# Autodesk Inventor assembly: WallBody
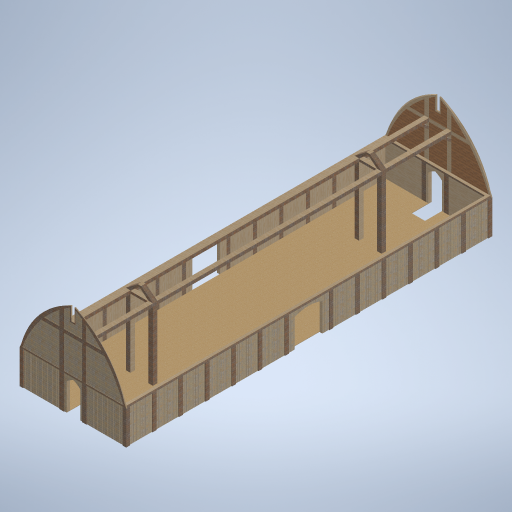
[picture p0: Inventor's stored thumbnail of the model, 512x512]
Saved by Autodesk Inventor 2024.2 (Build 282272000, 272)
## iProperties
Created: 2024-05-21
Part Number: WallBody
Document SubType Name: Assembly
Designer: LOSTER_1
Author: LOSTER_1
## Documents named in this file (62)
- C:\Users\LOSTER_1\OneDrive\桌面\school\senior\Inventor_Project\WALL\WallBody.iam
- C:\Users\LOSTER_1\OneDrive\桌面\school\senior\Inventor_Project\WALL\curve_front_wall_frame.ipt
- C:\Users\LOSTER_1\OneDrive\桌面\school\senior\Inventor_Project\WALL\top_wall_frame.ipt
- C:\Users\LOSTER_1\OneDrive\桌面\school\senior\Inventor_Project\WALL\front_wall_block01.ipt
- C:\Users\LOSTER_1\OneDrive\桌面\school\senior\Inventor_Project\WALL\front_wall_block02.ipt
- C:\Users\LOSTER_1\OneDrive\桌面\school\senior\Inventor_Project\WALL\front_wall_block03.ipt
- C:\Users\LOSTER_1\OneDrive\桌面\school\senior\Inventor_Project\WALL\front_wall_block04.ipt
- C:\Users\LOSTER_1\OneDrive\桌面\school\senior\Inventor_Project\WALL\front_wall_block01_MIR.ipt
- C:\Users\LOSTER_1\OneDrive\桌面\school\senior\Inventor_Project\WALL\front_wall_block02_MIR.ipt
- C:\Users\LOSTER_1\OneDrive\桌面\school\senior\Inventor_Project\WALL\front_wall_block03_MIR.ipt
- C:\Users\LOSTER_1\OneDrive\桌面\school\senior\Inventor_Project\WALL\front_wall_block04_MIR.ipt
- C:\Users\LOSTER_1\OneDrive\桌面\school\senior\Inventor_Project\WALL\curve_front_wall_frame_MIR.ipt
- C:\Users\LOSTER_1\OneDrive\桌面\school\senior\Inventor_Project\WALL\front_wall_block01_MIR1.ipt
- C:\Users\LOSTER_1\OneDrive\桌面\school\senior\Inventor_Project\WALL\front_wall_block02_MIR1.ipt
- C:\Users\LOSTER_1\OneDrive\桌面\school\senior\Inventor_Project\WALL\front_wall_block03_MIR1.ipt
- C:\Users\LOSTER_1\OneDrive\桌面\school\senior\Inventor_Project\WALL\front_wall_block04_MIR1.ipt
- C:\Users\LOSTER_1\OneDrive\桌面\school\senior\Inventor_Project\WALL\front_wall_block01_MIR_MIR.ipt
- C:\Users\LOSTER_1\OneDrive\桌面\school\senior\Inventor_Project\WALL\front_wall_block02_MIR_MIR.ipt
- C:\Users\LOSTER_1\OneDrive\桌面\school\senior\Inventor_Project\WALL\front_wall_block03_MIR_MIR.ipt
- C:\Users\LOSTER_1\OneDrive\桌面\school\senior\Inventor_Project\WALL\front_wall_block04_MIR_MIR.ipt
- C:\Users\LOSTER_1\OneDrive\桌面\school\senior\Inventor_Project\WALL\support_frame_01.ipt
- C:\Users\LOSTER_1\OneDrive\桌面\school\senior\Inventor_Project\WALL\support_frame_02.ipt
- C:\Users\LOSTER_1\OneDrive\桌面\school\senior\Inventor_Project\WALL\support_frame_02_MIR.ipt
- C:\Users\LOSTER_1\OneDrive\桌面\school\senior\Inventor_Project\WALL\support_frame_01_MIR.ipt
- C:\Users\LOSTER_1\OneDrive\桌面\school\senior\Inventor_Project\WALL\support_column_01.ipt
- C:\Users\LOSTER_1\OneDrive\桌面\school\senior\Inventor_Project\WALL\support_column_01_MIR.ipt
- C:\Users\LOSTER_1\OneDrive\桌面\school\senior\Inventor_Project\WALL\support_column_01_MIR1.ipt
- C:\Users\LOSTER_1\OneDrive\桌面\school\senior\Inventor_Project\WALL\support_column_01_MIR_MIR.ipt
- C:\Users\LOSTER_1\OneDrive\桌面\school\senior\Inventor_Project\WALL\support_column_02.ipt
- C:\Users\LOSTER_1\OneDrive\桌面\school\senior\Inventor_Project\WALL\support_column_02_MIR.ipt
- C:\Users\LOSTER_1\OneDrive\桌面\school\senior\Inventor_Project\WALL\support_column_02_MIR1.ipt
- C:\Users\LOSTER_1\OneDrive\桌面\school\senior\Inventor_Project\WALL\support_column_02_MIR_MIR.ipt
- C:\Users\LOSTER_1\OneDrive\桌面\school\senior\Inventor_Project\WALL\ribs\frame_rib_01.ipt
- C:\Users\LOSTER_1\OneDrive\桌面\school\senior\Inventor_Project\WALL\ribs\frame_rib_01_MIR.ipt
- C:\Users\LOSTER_1\OneDrive\桌面\school\senior\Inventor_Project\WALL\ribs\frame_rib_01_MIR1.ipt
- C:\Users\LOSTER_1\OneDrive\桌面\school\senior\Inventor_Project\WALL\ribs\frame_rib_01_MIR_MIR.ipt
- C:\Users\LOSTER_1\OneDrive\桌面\school\senior\Inventor_Project\WALL\ribs\frame_rib_02.ipt
- C:\Users\LOSTER_1\OneDrive\桌面\school\senior\Inventor_Project\WALL\ribs\frame_rib_02_MIR.ipt
- C:\Users\LOSTER_1\OneDrive\桌面\school\senior\Inventor_Project\WALL\ribs\frame_rib_02_MIR1.ipt
- C:\Users\LOSTER_1\OneDrive\桌面\school\senior\Inventor_Project\WALL\ribs\frame_rib_02_MIR_MIR.ipt
- C:\Users\LOSTER_1\OneDrive\桌面\school\senior\Inventor_Project\WALL\support_frame_03.ipt
- C:\Users\LOSTER_1\OneDrive\桌面\school\senior\Inventor_Project\WALL\support_frame_03_MIR.ipt
- C:\Users\LOSTER_1\OneDrive\桌面\school\senior\Inventor_Project\WALL\support_frame_03_MIR1.ipt
- C:\Users\LOSTER_1\OneDrive\桌面\school\senior\Inventor_Project\WALL\support_frame_03_MIR_MIR.ipt
- C:\Users\LOSTER_1\OneDrive\桌面\school\senior\Inventor_Project\WALL\normalized_wall_block\side_wall_block_01.ipt
- C:\Users\LOSTER_1\OneDrive\桌面\school\senior\Inventor_Project\WALL\normalized_wall_block\side_wall_block_02.ipt
- C:\Users\LOSTER_1\OneDrive\桌面\school\senior\Inventor_Project\WALL\normalized_wall_block\side_wall_block_01_MIR.ipt
- C:\Users\LOSTER_1\OneDrive\桌面\school\senior\Inventor_Project\WALL\support_column_01_MIR2.ipt
- C:\Users\LOSTER_1\OneDrive\桌面\school\senior\Inventor_Project\WALL\normalized_wall_block\side_wall_block_02_MIR.ipt
- C:\Users\LOSTER_1\OneDrive\桌面\school\senior\Inventor_Project\WALL\normalized_wall_block\side_wall_block_01_MIR1.ipt
- C:\Users\LOSTER_1\OneDrive\桌面\school\senior\Inventor_Project\WALL\support_column_01_MIR3.ipt
- C:\Users\LOSTER_1\OneDrive\桌面\school\senior\Inventor_Project\WALL\normalized_wall_block\side_wall_block_02_MIR1.ipt
- C:\Users\LOSTER_1\OneDrive\桌面\school\senior\Inventor_Project\WALL\normalized_wall_block\side_wall_block_01_MIR_MIR.ipt
- C:\Users\LOSTER_1\OneDrive\桌面\school\senior\Inventor_Project\WALL\support_column_01_MIR2_MIR.ipt
- C:\Users\LOSTER_1\OneDrive\桌面\school\senior\Inventor_Project\WALL\normalized_wall_block\side_wall_block_02_MIR_MIR.ipt
- C:\Users\LOSTER_1\OneDrive\桌面\school\senior\Inventor_Project\WALL\front_wall_block05.ipt
- C:\Users\LOSTER_1\OneDrive\桌面\school\senior\Inventor_Project\WALL\front_wall_block05_MIR.ipt
- C:\Users\LOSTER_1\OneDrive\桌面\school\senior\Inventor_Project\WALL\front_wall_block05_MIR1.ipt
- C:\Users\LOSTER_1\OneDrive\桌面\school\senior\Inventor_Project\WALL\front_wall_block05_MIR_MIR.ipt
- C:\Users\LOSTER_1\OneDrive\桌面\school\senior\Inventor_Project\WALL\front_wall_block06.ipt
- C:\Users\LOSTER_1\OneDrive\桌面\school\senior\Inventor_Project\FLOOR\inside_floor.ipt
- C:\Users\LOSTER_1\OneDrive\桌面\school\senior\Inventor_Project\WALL\front_wall_block06_MIR1.ipt
## Components (102 placed, 61 different names)
1. curve_front_wall_frame:1 — Flush:1, Mate:1, Mate:2, Flush:2, Mate:3, Mate:4, Mate:5, Mate:7, Mate:8, Mate:9, Mate:18
2. top_wall_frame:1 — Mate:1, Mate:2, Mate:6, Mate:10, Mate:24, Mate:35, Mate:36, Mate:37, Mate:39, Mate:41, Mate:43, Mate:45, Mate:47, Mate:49, Mate:51, Mate:53, Mate:55, Mate:57, Mate:59, Mate:97, Mate:99
3. front_wall_block01:1 — Mate:3, Mate:4
4. front_wall_block02:1 — Mate:5, Mate:6
5. front_wall_block03:1 — Mate:7, Mate:8
6. front_wall_block04:1 — Mate:9, Mate:10
7. front_wall_block01_MIR:1
8. front_wall_block02_MIR:1 — Mate:19, Mate:20
9. front_wall_block03_MIR:1
10. front_wall_block04_MIR:1
11. curve_front_wall_frame_MIR:1 — Mate:11, Mate:12, Mate:13, Mate:14, Mate:15, Mate:16, Mate:17, Mate:25, Mate:26, Mate:27, Mate:28
12. front_wall_block01_MIR1:1 — Mate:12, Mate:13
13. front_wall_block02_MIR1:1 — Mate:14
14. front_wall_block03_MIR1:1 — Mate:15, Mate:16
15. front_wall_block04_MIR1:1 — Mate:17
16. front_wall_block01_MIR_MIR:1
17. front_wall_block02_MIR_MIR:1
18. front_wall_block03_MIR_MIR:1
19. front_wall_block04_MIR_MIR:1
20. support_frame_01:1 — Mate:18, Mate:19, Mate:20, Mate:21, Mate:22, Mate:23
21. support_frame_02:1 — Mate:21, Mate:22, Mate:23
22. support_frame_02_MIR:1
23. support_frame_01_MIR:1 — Mate:29, Mate:30, Mate:31, Mate:32, Mate:33, Mate:34
24. support_column_01:1 — Mate:24, Mate:25, Mate:26
25. support_column_01_MIR:1
26. support_column_01_MIR1:1
27. support_column_01_MIR_MIR:1
28. support_column_02:1 — Mate:27, Mate:28, Mate:100
29. support_column_02_MIR:1
30. support_column_02_MIR1:1
31. support_column_02_MIR_MIR:1
32. frame_rib_01:1 — Mate:29, Mate:30
33. frame_rib_01_MIR:1
34. frame_rib_01_MIR1:1
35. frame_rib_01_MIR_MIR:1
36. frame_rib_02:1 — Mate:31, Mate:32
37. frame_rib_02_MIR:1
38. frame_rib_02_MIR1:1
39. frame_rib_02_MIR_MIR:1
40. support_frame_03:1 — Mate:33, Mate:34
41. support_frame_03_MIR:1
42. support_frame_03_MIR1:1
43. support_frame_03_MIR_MIR:1
44. side_wall_block_01:1 — Mate:35, Mate:36, Mate:38, Mate:98
45. support_column_01:2 — Mate:37, Mate:38, Mate:40
46. side_wall_block_01:2 — Mate:39, Mate:40, Mate:42
47. support_column_01:3 — Mate:41, Mate:42, Mate:44
48. side_wall_block_01:3 — Mate:43, Mate:44, Mate:46
49. support_column_01:4 — Mate:45, Mate:46, Mate:48
50. side_wall_block_01:4 — Mate:47, Mate:48, Mate:50
51. support_column_01:5 — Mate:49, Mate:50, Mate:52
52. side_wall_block_01:5 — Mate:51, Mate:52, Mate:54
53. support_column_01:6 — Mate:53, Mate:54, Mate:56
54. side_wall_block_01:6 — Mate:55, Mate:56, Mate:58
55. support_column_01:7 — Mate:57, Mate:58, Mate:60
56. side_wall_block_02:1 — Mate:59, Mate:60
57. side_wall_block_01_MIR:1 — Mate:61
58. support_column_01_MIR2:1 — Mate:61, Mate:62
59. side_wall_block_01_MIR:2 — Mate:62, Mate:63
60. support_column_01_MIR2:2 — Mate:63, Mate:64
61. side_wall_block_01_MIR:3 — Mate:64, Mate:65
62. support_column_01_MIR2:3 — Mate:65, Mate:66
63. side_wall_block_01_MIR:4 — Mate:66, Mate:67
64. support_column_01_MIR2:4 — Mate:67, Mate:68
65. side_wall_block_01_MIR:5 — Mate:68, Mate:69
66. support_column_01_MIR2:5 — Mate:69, Mate:70
67. side_wall_block_01_MIR:6 — Mate:70, Mate:71
68. support_column_01_MIR2:6 — Mate:71, Mate:72
69. side_wall_block_02_MIR:1 — Mate:72
70. side_wall_block_01_MIR1:1 — Mate:73
71. support_column_01_MIR3:1 — Mate:73, Mate:74
72. side_wall_block_01_MIR1:2 — Mate:74, Mate:75
73. support_column_01_MIR3:2 — Mate:75, Mate:76
74. side_wall_block_01_MIR1:3 — Mate:76, Mate:77
75. support_column_01_MIR3:3 — Mate:77, Mate:78
76. side_wall_block_01_MIR1:4 — Mate:78, Mate:79
77. support_column_01_MIR3:4 — Mate:79, Mate:80
78. side_wall_block_01_MIR1:5 — Mate:80, Mate:81
79. support_column_01_MIR3:5 — Mate:81, Mate:82
80. side_wall_block_01_MIR1:6 — Mate:82, Mate:83
81. support_column_01_MIR3:6 — Mate:83, Mate:84
82. side_wall_block_02_MIR1:1 — Mate:84
83. side_wall_block_01_MIR_MIR:1 — Mate:85
84. support_column_01_MIR2_MIR:1 — Mate:85, Mate:86
85. side_wall_block_01_MIR_MIR:2 — Mate:86, Mate:87
86. support_column_01_MIR2_MIR:2 — Mate:87, Mate:88
87. side_wall_block_01_MIR_MIR:3 — Mate:88, Mate:89
88. support_column_01_MIR2_MIR:3 — Mate:89, Mate:90
89. side_wall_block_01_MIR_MIR:4 — Mate:90, Mate:91
90. support_column_01_MIR2_MIR:4 — Mate:91, Mate:92
91. side_wall_block_01_MIR_MIR:5 — Mate:92, Mate:93
92. support_column_01_MIR2_MIR:5 — Mate:93, Mate:94
93. side_wall_block_01_MIR_MIR:6 — Mate:94, Mate:95
94. support_column_01_MIR2_MIR:6 — Mate:95, Mate:96
95. side_wall_block_02_MIR_MIR:1 — Mate:96
96. front_wall_block05:1 — Mate:97, Mate:98
97. front_wall_block05_MIR:1 — Mate:101
98. front_wall_block05_MIR1:1
99. front_wall_block05_MIR_MIR:1
100. front_wall_block06:1 — Mate:99, Mate:100
101. inside_floor:1 — Mate:101
102. front_wall_block06_MIR1:1
## Relationships (103: Mate 101, Flush 2)
- Flush:1 (16151 mm): curve_front_wall_frame:1
- Mate:1: curve_front_wall_frame:1 ↔ top_wall_frame:1
- Mate:2: curve_front_wall_frame:1 ↔ top_wall_frame:1
- Flush:2 (150 mm): curve_front_wall_frame:1
- Mate:3: curve_front_wall_frame:1 ↔ front_wall_block01:1
- Mate:4: curve_front_wall_frame:1 ↔ front_wall_block01:1
- Mate:5: curve_front_wall_frame:1 ↔ front_wall_block02:1
- Mate:6: top_wall_frame:1 ↔ front_wall_block02:1
- Mate:7: curve_front_wall_frame:1 ↔ front_wall_block03:1
- Mate:8: curve_front_wall_frame:1 ↔ front_wall_block03:1
- Mate:9: curve_front_wall_frame:1 ↔ front_wall_block04:1
- Mate:10: top_wall_frame:1 ↔ front_wall_block04:1
- Mate:11 (16151 mm): curve_front_wall_frame_MIR:1
- Mate:12: curve_front_wall_frame_MIR:1 ↔ front_wall_block01_MIR1:1
- Mate:13: curve_front_wall_frame_MIR:1 ↔ front_wall_block01_MIR1:1
- Mate:14: curve_front_wall_frame_MIR:1 ↔ front_wall_block02_MIR1:1
- Mate:15: curve_front_wall_frame_MIR:1 ↔ front_wall_block03_MIR1:1
- Mate:16: curve_front_wall_frame_MIR:1 ↔ front_wall_block03_MIR1:1
- Mate:17: curve_front_wall_frame_MIR:1 ↔ front_wall_block04_MIR1:1
- Mate:18: curve_front_wall_frame:1 ↔ support_frame_01:1
- Mate:19: front_wall_block02_MIR:1 ↔ support_frame_01:1
- Mate:20: front_wall_block02_MIR:1 ↔ support_frame_01:1
- Mate:21: support_frame_01:1 ↔ support_frame_02:1
- Mate:22: support_frame_01:1 ↔ support_frame_02:1
- Mate:23: support_frame_01:1 ↔ support_frame_02:1
- Mate:24: top_wall_frame:1 ↔ support_column_01:1
- Mate:25: curve_front_wall_frame_MIR:1 ↔ support_column_01:1
- Mate:26: curve_front_wall_frame_MIR:1 ↔ support_column_01:1
- Mate:27: curve_front_wall_frame_MIR:1 ↔ support_column_02:1
- Mate:28: curve_front_wall_frame_MIR:1 ↔ support_column_02:1
- Mate:29: support_frame_01_MIR:1 ↔ frame_rib_01:1
- Mate:30: support_frame_01_MIR:1 ↔ frame_rib_01:1
- Mate:31: support_frame_01_MIR:1 ↔ frame_rib_02:1
- Mate:32: support_frame_01_MIR:1 ↔ frame_rib_02:1
- Mate:33: support_frame_01_MIR:1 ↔ support_frame_03:1
- Mate:34: support_frame_01_MIR:1 ↔ support_frame_03:1
- Mate:35: top_wall_frame:1 ↔ side_wall_block_01:1
- Mate:36: top_wall_frame:1 ↔ side_wall_block_01:1
- Mate:37: top_wall_frame:1 ↔ support_column_01:2
- Mate:38: side_wall_block_01:1 ↔ support_column_01:2
- Mate:39: top_wall_frame:1 ↔ side_wall_block_01:2
- Mate:40: support_column_01:2 ↔ side_wall_block_01:2
- Mate:41: top_wall_frame:1 ↔ support_column_01:3
- Mate:42: side_wall_block_01:2 ↔ support_column_01:3
- Mate:43: top_wall_frame:1 ↔ side_wall_block_01:3
- Mate:44: support_column_01:3 ↔ side_wall_block_01:3
- Mate:45: top_wall_frame:1 ↔ support_column_01:4
- Mate:46: side_wall_block_01:3 ↔ support_column_01:4
- Mate:47: top_wall_frame:1 ↔ side_wall_block_01:4
- Mate:48: support_column_01:4 ↔ side_wall_block_01:4
- Mate:49: top_wall_frame:1 ↔ support_column_01:5
- Mate:50: side_wall_block_01:4 ↔ support_column_01:5
- Mate:51: top_wall_frame:1 ↔ side_wall_block_01:5
- Mate:52: support_column_01:5 ↔ side_wall_block_01:5
- Mate:53: top_wall_frame:1 ↔ support_column_01:6
- Mate:54: side_wall_block_01:5 ↔ support_column_01:6
- Mate:55: top_wall_frame:1 ↔ side_wall_block_01:6
- Mate:56: support_column_01:6 ↔ side_wall_block_01:6
- Mate:57: top_wall_frame:1 ↔ support_column_01:7
- Mate:58: side_wall_block_01:6 ↔ support_column_01:7
- Mate:59: top_wall_frame:1 ↔ side_wall_block_02:1
- Mate:60: support_column_01:7 ↔ side_wall_block_02:1
- Mate:61: side_wall_block_01_MIR:1 ↔ support_column_01_MIR2:1
- Mate:62: support_column_01_MIR2:1 ↔ side_wall_block_01_MIR:2
- Mate:63: side_wall_block_01_MIR:2 ↔ support_column_01_MIR2:2
- Mate:64: support_column_01_MIR2:2 ↔ side_wall_block_01_MIR:3
- Mate:65: side_wall_block_01_MIR:3 ↔ support_column_01_MIR2:3
- Mate:66: support_column_01_MIR2:3 ↔ side_wall_block_01_MIR:4
- Mate:67: side_wall_block_01_MIR:4 ↔ support_column_01_MIR2:4
- Mate:68: support_column_01_MIR2:4 ↔ side_wall_block_01_MIR:5
- Mate:69: side_wall_block_01_MIR:5 ↔ support_column_01_MIR2:5
- Mate:70: support_column_01_MIR2:5 ↔ side_wall_block_01_MIR:6
- Mate:71: side_wall_block_01_MIR:6 ↔ support_column_01_MIR2:6
- Mate:72: support_column_01_MIR2:6 ↔ side_wall_block_02_MIR:1
- Mate:73: side_wall_block_01_MIR1:1 ↔ support_column_01_MIR3:1
- Mate:74: support_column_01_MIR3:1 ↔ side_wall_block_01_MIR1:2
- Mate:75: side_wall_block_01_MIR1:2 ↔ support_column_01_MIR3:2
- Mate:76: support_column_01_MIR3:2 ↔ side_wall_block_01_MIR1:3
- Mate:77: side_wall_block_01_MIR1:3 ↔ support_column_01_MIR3:3
- Mate:78: support_column_01_MIR3:3 ↔ side_wall_block_01_MIR1:4
- Mate:79: side_wall_block_01_MIR1:4 ↔ support_column_01_MIR3:4
- Mate:80: support_column_01_MIR3:4 ↔ side_wall_block_01_MIR1:5
- Mate:81: side_wall_block_01_MIR1:5 ↔ support_column_01_MIR3:5
- Mate:82: support_column_01_MIR3:5 ↔ side_wall_block_01_MIR1:6
- Mate:83: side_wall_block_01_MIR1:6 ↔ support_column_01_MIR3:6
- Mate:84: support_column_01_MIR3:6 ↔ side_wall_block_02_MIR1:1
- Mate:85: side_wall_block_01_MIR_MIR:1 ↔ support_column_01_MIR2_MIR:1
- Mate:86: support_column_01_MIR2_MIR:1 ↔ side_wall_block_01_MIR_MIR:2
- Mate:87: side_wall_block_01_MIR_MIR:2 ↔ support_column_01_MIR2_MIR:2
- Mate:88: support_column_01_MIR2_MIR:2 ↔ side_wall_block_01_MIR_MIR:3
- Mate:89: side_wall_block_01_MIR_MIR:3 ↔ support_column_01_MIR2_MIR:3
- Mate:90: support_column_01_MIR2_MIR:3 ↔ side_wall_block_01_MIR_MIR:4
- Mate:91: side_wall_block_01_MIR_MIR:4 ↔ support_column_01_MIR2_MIR:4
- Mate:92: support_column_01_MIR2_MIR:4 ↔ side_wall_block_01_MIR_MIR:5
- Mate:93: side_wall_block_01_MIR_MIR:5 ↔ support_column_01_MIR2_MIR:5
- Mate:94: support_column_01_MIR2_MIR:5 ↔ side_wall_block_01_MIR_MIR:6
- Mate:95: side_wall_block_01_MIR_MIR:6 ↔ support_column_01_MIR2_MIR:6
- Mate:96: support_column_01_MIR2_MIR:6 ↔ side_wall_block_02_MIR_MIR:1
- Mate:97: top_wall_frame:1 ↔ front_wall_block05:1
- Mate:98: side_wall_block_01:1 ↔ front_wall_block05:1
- Mate:99: top_wall_frame:1 ↔ front_wall_block06:1
- Mate:100: support_column_02:1 ↔ front_wall_block06:1
- Mate:101: front_wall_block05_MIR:1 ↔ inside_floor:1
